# Autodesk Inventor assembly: pasekturbonowy
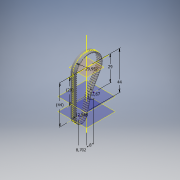
[picture p0: Inventor's stored thumbnail of the model, 180x180]
Saved by Autodesk Inventor 2019 (Build 230136000, 136)
## iProperties
Created: 2020-08-27
Part Number: pasekturbonowy
Document SubType Name: Assembly
Designer: estee
Author: estee
## Documents named in this file (4)
- C:\Users\estee\OneDrive\Pulpit\estere\1\MUM\nowygit\Mechanika\Moduł obrotu RET Estera\projejt\pasekturbonowy.iam
- C:\Users\estee\OneDrive\Pulpit\estere\1\MUM\nowygit\Mechanika\Moduł obrotu RET Estera\projejt\czesc1paska.ipt
- C:\Users\estee\OneDrive\Pulpit\estere\1\MUM\nowygit\Mechanika\Moduł obrotu RET Estera\projejt\zab.ipt
- C:\Users\estee\OneDrive\Pulpit\estere\1\MUM\nowygit\Mechanika\Moduł obrotu RET Estera\projejt\czesc2paska.ipt
## Components (82 placed, 3 different names)
1. czesc1paska:1 — Flush:1, Flush:2, Flush:3, Mate:1, Mate:2, Mate:3, Mate:5, Angle:2
2. czesc2paska:1 — Mate:6, Mate:7, Flush:4
3. zab:1 — Mate:3, Mate:4, Angle:1
4. zab:2
5. zab:3
6. zab:4
7. zab:5
8. zab:6
9. zab:7
10. zab:8
11. zab:9
12. zab:10
13. zab:11
14. zab:12
15. zab:13
16. zab:14
17. zab:15
18. zab:16
19. zab:17
20. zab:18
21. zab:19
22. zab:20
23. zab:21
24. zab:22
25. zab:23
26. zab:24
27. zab:25
28. zab:26
29. zab:27
30. zab:28
31. zab:29
32. zab:30
33. zab:31
34. zab:32
35. zab:33
36. zab:34
37. zab:35
38. zab:36
39. zab:37
40. zab:38
41. zab:39
42. zab:40
43. zab:41
44. zab:42
45. zab:43
46. zab:44
47. zab:45
48. zab:46
49. zab:47
50. zab:48
51. zab:49
52. zab:50
53. zab:51
54. zab:52
55. zab:53
56. zab:54
57. zab:55
58. zab:56
59. zab:57
60. zab:58
61. zab:59
62. zab:60
63. zab:61
64. zab:62
65. zab:63
66. zab:64
67. zab:65
68. zab:66
69. zab:67
70. zab:68
71. zab:69
72. zab:70
73. zab:71
74. zab:72
75. zab:73
76. zab:74
77. zab:75
78. zab:76
79. zab:77
80. zab:78
81. zab:79
82. zab:80
## Component patterns: (80 elements, first: zab:1)
## Relationships (13: Mate 7, Flush 4, Angle 2)
- Flush:1: czesc1paska:1
- Flush:2: czesc1paska:1
- Flush:3: czesc1paska:1
- Mate:1 (-44 mm): czesc1paska:1
- Mate:2 (-29 mm): czesc1paska:1
- Mate:3: czesc1paska:1 ↔ zab:1
- Mate:4 (3 mm): zab:1
- Angle:1 (0 deg): zab:1
- Mate:5: czesc1paska:1
- Angle:2 (0 deg): czesc1paska:1
- Mate:6: czesc2paska:1
- Mate:7: czesc2paska:1
- Flush:4: czesc2paska:1
